# Autodesk Inventor assembly: ASSEMBLY_Solenoid_Actuator
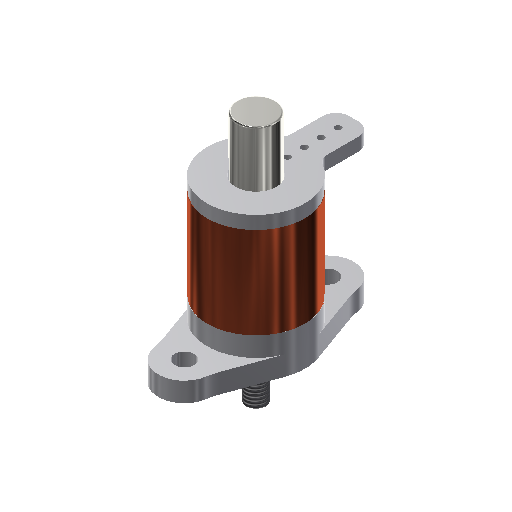
[picture p0: Inventor's stored thumbnail of the model, 512x512]
Saved by Autodesk Inventor 2026.1 (Build 301233000, 233)
## iProperties
Created: 2018-06-14
Part Number: ASSEMBLY_Solenoid_Actuator
Document SubType Name: Assembly
Designer: Andrzej
Author: Andrzej
## Documents named in this file (6)
- C:\Users\Andrzej\OneDrive\_DRIVE_SYNCH_FILES\__ BYTECHLAB PROJECTS\MLTDIS - SMD Parts Sorting Machine\MCAD\1_REV1\ASSEMBLY_MEASUREMENT_RAIL_REVA\ASSEMBLY_MAIN_REVA\ASSEMBLY_Solenoid_Actuator.iam
- C:\Users\Andrzej\OneDrive\_DRIVE_SYNCH_FILES\__ BYTECHLAB PROJECTS\MLTDIS - SMD Parts Sorting Machine\MCAD\1_REV1\ASSEMBLY_MEASUREMENT_RAIL_REVA\ASSEMBLY_MAIN_REVA\3DP_ABS_Solenoid_Actuator_Body.ipt
- C:\Users\Andrzej\OneDrive\_DRIVE_SYNCH_FILES\__ BYTECHLAB PROJECTS\MLTDIS - SMD Parts Sorting Machine\MCAD\1_REV1\ASSEMBLY_MEASUREMENT_RAIL_REVA\__COTS_PARTS\COTS_GENERIC_Solenoid_Actuator_Coil.ipt
- C:\Users\Andrzej\OneDrive\_DRIVE_SYNCH_FILES\__ BYTECHLAB PROJECTS\MLTDIS - SMD Parts Sorting Machine\MCAD\1_REV1\ASSEMBLY_MEASUREMENT_RAIL_REVA\__COTS_PARTS\COTS_GENERIC_6x15mm_Neodymium_Magnet.ipt
- C:\Users\Andrzej\OneDrive\_DRIVE_SYNCH_FILES\__ BYTECHLAB PROJECTS\MLTDIS - SMD Parts Sorting Machine\MCAD\1_REV1\ASSEMBLY_MEASUREMENT_RAIL_REVA\__COTS_PARTS\COTS_GENERIC_Solenoid_Actuator_Push_Rod_M3.ipt
- C:\Users\Andrzej\OneDrive\_DRIVE_SYNCH_FILES\__ BYTECHLAB PROJECTS\MLTDIS - SMD Parts Sorting Machine\MCAD\1_REV1\ASSEMBLY_MEASUREMENT_RAIL_REVA\ASSEMBLY_MAIN_REVA\3DP_ABS_Solenoid_Actuator_Offset_Spacer.ipt
## Components (5 placed, 5 different names)
1. 3DP_ABS_Solenoid_Actuator_Body:1 — Mate:1, Mate:2, Mate:5, Mate:6
2. COTS_GENERIC_Solenoid_Actuator_Coil:1 — Mate:1, Mate:2
3. COTS_GENERIC_6x15mm_Neodymium_Magnet:1 — Mate:7, Mate:8
4. COTS_GENERIC_Solenoid_Actuator_Push_Rod_M3:1 — Mate:3, Mate:4, Mate:5, Mate:7, Mate:8
5. 3DP_ABS_Solenoid_Actuator_Offset_Spacer:1 — Mate:3, Mate:4, Mate:6
## Relationships (8: Mate 8)
- Mate:1: 3DP_ABS_Solenoid_Actuator_Body:1 ↔ COTS_GENERIC_Solenoid_Actuator_Coil:1
- Mate:2: 3DP_ABS_Solenoid_Actuator_Body:1 ↔ COTS_GENERIC_Solenoid_Actuator_Coil:1
- Mate:3: COTS_GENERIC_Solenoid_Actuator_Push_Rod_M3:1 ↔ 3DP_ABS_Solenoid_Actuator_Offset_Spacer:1
- Mate:4: COTS_GENERIC_Solenoid_Actuator_Push_Rod_M3:1 ↔ 3DP_ABS_Solenoid_Actuator_Offset_Spacer:1
- Mate:5: 3DP_ABS_Solenoid_Actuator_Body:1 ↔ COTS_GENERIC_Solenoid_Actuator_Push_Rod_M3:1
- Mate:6 (1 mm): 3DP_ABS_Solenoid_Actuator_Body:1 ↔ 3DP_ABS_Solenoid_Actuator_Offset_Spacer:1
- Mate:7: COTS_GENERIC_6x15mm_Neodymium_Magnet:1 ↔ COTS_GENERIC_Solenoid_Actuator_Push_Rod_M3:1
- Mate:8: COTS_GENERIC_6x15mm_Neodymium_Magnet:1 ↔ COTS_GENERIC_Solenoid_Actuator_Push_Rod_M3:1
